# Autodesk Inventor assembly: Assembly8
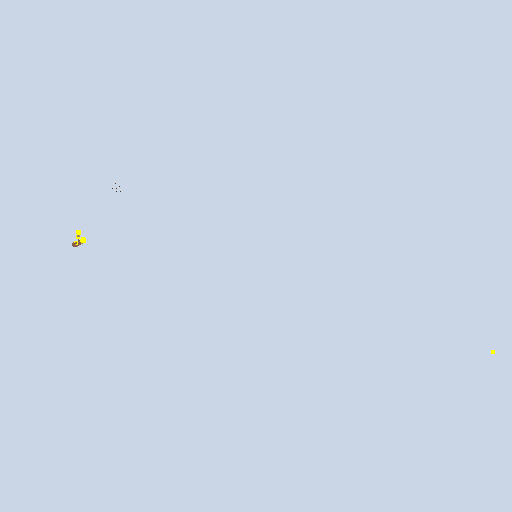
[picture p0: Inventor's stored thumbnail of the model, 512x512]
Saved by Autodesk Inventor 2024.1 (Build 281209000, 209)
## iProperties
Created: 2023-11-10
Part Number: Assembly8
Document SubType Name: Assembly
Designer: luvag
Author: luvag
## Documents named in this file (3)
- C:\Users\luvag\Desktop\Assembly8.iam
- C:\Users\luvag\Desktop\Cannon.ipt
- C:\Users\luvag\Desktop\Assembly3.iam
## Components (2 placed, 2 different names)
1. Cannon:1
2. Assembly3:1 [sub-assembly]
## Relationships (2: Mate 2)
- [Mate]: Cannon:1 ↔ Assembly3:1
- [Mate]: Cannon:1 ↔ Assembly3:1
